# Autodesk Inventor assembly: (Unsaved)
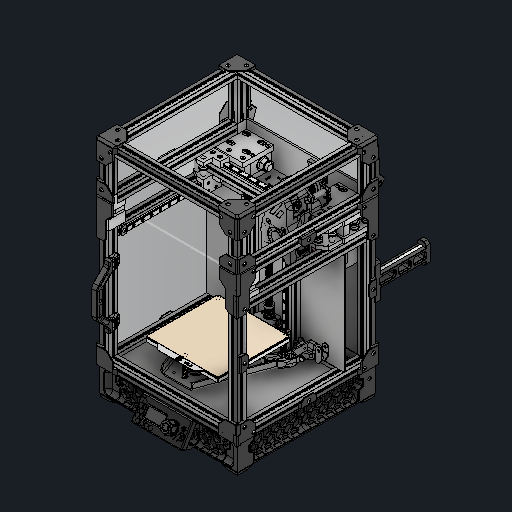
[picture p0: Inventor's stored thumbnail of the model, 512x512]
Saved by Autodesk Inventor 2025.1 (Build 291241020, 241B)
## iProperties
Created: 2025-05-09
Part Number: (Unsaved)
Document SubType Name: Assembly
Designer: AdminForWorker
Title: Voron 0 v2
Author: AdminForWorker
## Documents named in this file (19)
- C:\Users\Joshua Eah\Documents\Voron 0.2\CAD\Master Assembly\Voron 0.iam
- C:\Users\Joshua Eah\Documents\Voron 0.2\CAD\Master Assembly\Frame\Frame.iam
- C:\Users\Joshua Eah\Documents\Voron 0.2\CAD\Master Assembly\Skirt\Skirts.iam
- C:\Users\Joshua Eah\Documents\Voron 0.2\CAD\Master Assembly\Panels\Panels & Clips.iam
- C:\Users\Joshua Eah\Documents\Voron 0.2\CAD\Master Assembly\Frame\Extrusion Tophat.iam
- C:\Users\Joshua Eah\Documents\Voron 0.2\CAD\Master Assembly\Electronics\Electronics.iam
- C:\Users\Joshua Eah\Documents\Voron 0.2\CAD\Master Assembly\Extras\Filament Spool.iam
- C:\Users\Joshua Eah\Documents\Voron 0.2\CAD\Master Assembly\Z Axis\Bed Assembly.iam
- C:\Users\Joshua Eah\Documents\Voron 0.2\CAD\Master Assembly\Z Axis\Z Motor Assembly.iam
- C:\Users\Joshua Eah\Documents\Voron 0.2\CAD\Master Assembly\Frame\Subassemblies\Z Extrusion Right.iam
- Z Extrusion Right.iam
- C:\Users\Joshua Eah\Documents\Voron 0.2\CAD\Master Assembly\Frame\Subassemblies\Z Extrusion Left.iam
- C:\Users\Joshua Eah\Documents\Voron 0.2\CAD\Master Assembly\Linear Rail\Parts\MGN7H Carriage.ipt
- C:\Users\Joshua Eah\Documents\Voron 0.2\CAD\Master Assembly\Motion\Belts\Belts.iam
- C:\Users\Joshua Eah\Documents\Voron 0.2\CAD\Master Assembly\Motion\AB Drives\A_B Drives.iam
- C:\Users\Joshua Eah\Documents\Voron 0.2\CAD\Master Assembly\Motion\Idlers\Idlers.iam
- C:\Users\Joshua Eah\Documents\Voron 0.2\CAD\Master Assembly\X Axis\X Axis.iam
- C:\Users\Joshua Eah\Documents\Voron 0.2\CAD\Master Assembly\Toolhead\Mini Stealthburner.iam
- C:\Users\Joshua Eah\Documents\Voron 0.2\CAD\Master Assembly\Panels\Door Assembly.iam
## Components (21 placed, 21 different names)
1. Frame:1 [sub-assembly] — Flush:3, Angle:1, Mate:4, Cylindrical:5, Cylindrical:6, Cylindrical:7, Cylindrical:8
2. Belts:1 [sub-assembly]
3. A/B Drives:1 [sub-assembly]
4. Idlers:1 [sub-assembly]
5. X Axis:1 [sub-assembly] — Mate:6, Mate:7, Mate:8, Mate:9, Mate:10, Cylindrical:9, Cylindrical:10
6. MGN7H X Carriage:1 — Cylindrical:9, Cylindrical:10, Insert:5, Insert:6
7. Mini Stealthburner:1 [sub-assembly] — Insert:5, Insert:6
8. MGN7H Y Left Carriage:1 — Cylindrical:5, Cylindrical:6, Mate:6, Mate:8, Mate:9
9. MGN7H Y Right Carriage:1 — Cylindrical:7, Cylindrical:8, Mate:7, Mate:10
10. Bed Assembly:1 [sub-assembly] — Mate:1, Insert:1, Insert:2, Insert:3, Insert:4
11. Z Motor Assembly:1 [sub-assembly] — Mate:1, Flush:3, Angle:1
12. Z Extrusion Right:1 [sub-assembly] — Cylindrical:3, Cylindrical:4
13. Z Extrusion Left:1 [sub-assembly] — Cylindrical:1, Cylindrical:2, Mate:4
14. MGN7H Z Left Carriage:1 — Cylindrical:1, Cylindrical:2, Insert:2, Insert:3
15. MGN7H Z Right Carriage:1 — Cylindrical:3, Cylindrical:4, Insert:1, Insert:4
16. Skirts:1 [sub-assembly]
17. Panels & Clips:1 [sub-assembly] — Rotational:1, Rotational:2
18. Door Assembly:1 [sub-assembly] — Rotational:1
19. Extrusion Tophat:1 [sub-assembly] — Rotational:2
20. Electronics:1 [sub-assembly]
21. Filament Spool:1 [sub-assembly]
## Relationships (32: CylindricalJoint 10, Mate 9, Insert 6, Flush 4, RevoluteJoint 2, Angle 1)
- Mate:1: Bed Assembly:1 ↔ Z Motor Assembly:1
- [Mate]: Frame:1 ↔ Z Extrusion Right:1
- [Mate]: Frame:1 ↔ Z Extrusion Left:1
- [Flush]: Frame:1 ↔ Z Extrusion Right:1
- [Flush]: Frame:1 ↔ Z Extrusion Left:1
- Cylindrical:1: Z Extrusion Left:1 ↔ MGN7H Z Left Carriage:1
- Cylindrical:2: Z Extrusion Left:1 ↔ MGN7H Z Left Carriage:1
- Cylindrical:3: Z Extrusion Right:1 ↔ MGN7H Z Right Carriage:1
- Cylindrical:4: Z Extrusion Right:1 ↔ MGN7H Z Right Carriage:1
- Insert:1: Bed Assembly:1 ↔ MGN7H Z Right Carriage:1
- Insert:2: Bed Assembly:1 ↔ MGN7H Z Left Carriage:1
- Insert:3: Bed Assembly:1 ↔ MGN7H Z Left Carriage:1
- Insert:4: Bed Assembly:1 ↔ MGN7H Z Right Carriage:1
- Flush:3: Frame:1 ↔ Z Motor Assembly:1
- Angle:1 (0 deg): Frame:1 ↔ Z Motor Assembly:1
- Mate:4 (58 mm): Frame:1 ↔ Z Extrusion Left:1
- [Flush]: Bed Assembly:1 ↔ Z Extrusion Right:1
- Cylindrical:5: Frame:1 ↔ MGN7H Y Left Carriage:1
- Cylindrical:6: Frame:1 ↔ MGN7H Y Left Carriage:1
- Cylindrical:7: Frame:1 ↔ MGN7H Y Right Carriage:1
- Cylindrical:8: Frame:1 ↔ MGN7H Y Right Carriage:1
- Mate:6: X Axis:1 ↔ MGN7H Y Left Carriage:1
- Mate:7: X Axis:1 ↔ MGN7H Y Right Carriage:1
- Mate:8: X Axis:1 ↔ MGN7H Y Left Carriage:1
- Mate:9: X Axis:1 ↔ MGN7H Y Left Carriage:1
- Mate:10: X Axis:1 ↔ MGN7H Y Right Carriage:1
- Cylindrical:9: X Axis:1 ↔ MGN7H X Carriage:1
- Cylindrical:10: X Axis:1 ↔ MGN7H X Carriage:1
- Insert:5: MGN7H X Carriage:1 ↔ Mini Stealthburner:1
- Insert:6: MGN7H X Carriage:1 ↔ Mini Stealthburner:1
- Rotational:1 [RevoluteJoint]: Panels & Clips:1 ↔ Door Assembly:1
- Rotational:2 [RevoluteJoint]: Panels & Clips:1 ↔ Extrusion Tophat:1
